# Autodesk Inventor assembly: Assembly1
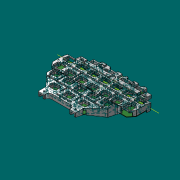
[picture p0: Inventor's stored thumbnail of the model, 180x180]
Saved by Autodesk Inventor 2018 (Build 220112000, 112)
## iProperties
Created: 2021-10-17
Part Number: Assembly1
Material: 一般
Document SubType Name: Assembly
Designer: gisen
Author: gisen
## Documents named in this file (5)
- C:\Users\gisen\Documents\CAD\inventor\git\logicool_g13_mod\mechanical_key\inventor\Assembly1.iam
- C:\Users\gisen\Documents\CAD\inventor\git\logicool_g13_mod\mechanical_key\inventor\plastic_mount2.ipt
- C:\Users\gisen\Documents\CAD\inventor\git\logicool_g13_mod\mechanical_key\inventor\pcb_top.ipt
- C:\Users\gisen\Documents\CAD\inventor\git\logicool_g13_mod\mechanical_key\inventor\pcb_middle.ipt
- C:\Users\gisen\Documents\CAD\inventor\git\logicool_g13_mod\mechanical_key\inventor\Part2.ipt
## Components (4 placed, 4 different names)
1. plastic_mount2:1 — フラッシュ:1, フラッシュ:2, フラッシュ:3
2. pcb_top:1 — フラッシュ:1
3. pcb_middle:1 — フラッシュ:2
4. Part2:1 — フラッシュ:4
## Relationships (4: Flush 4)
- フラッシュ:1 [Flush]: plastic_mount2:1 ↔ pcb_top:1
- フラッシュ:2 [Flush]: plastic_mount2:1 ↔ pcb_middle:1
- フラッシュ:3 [Flush] (0.8 mm): plastic_mount2:1
- フラッシュ:4 [Flush]: Part2:1
